# Autodesk Inventor assembly: 00_044_THORAX_YAW_R1
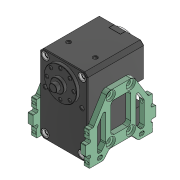
[picture p0: Inventor's stored thumbnail of the model, 180x180]
Saved by Autodesk Inventor 2021.2 (Build 252289000, 289)
## iProperties
Created: 2018-08-06
Part Number: 00_044_THORAX_YAW_R1
Material: 一般
Document SubType Name: Assembly
Designer: student
Mass: 66.6076 g
Surface Area: 177.769 cm^2
Volume: 47.0989 cm^3
Density: 1.41421 g/cm^3
Author: student
## Documents named in this file (4)
- C:\Workspace\HaptHexa\Hardware\Inventor\00_044_THORAX_YAW_R1.iam
- C:\Workspace\HaptHexa\Hardware\Inventor\16_045_THORAX_YAW_FRAME1_R1.ipt
- C:\Workspace\HaptHexa\Hardware\Inventor\20_001_DYNAMIXEL_X430_R1.ipt
- C:\Workspace\HaptHexa\Hardware\Inventor\16_029_X430_FREE_HORN_R1.ipt
## Components (4 placed, 3 different names)
1. yaw_servo_side:1 — Mate:5, Mate:6, Mate:7
2. 20_001_DYNAMIXEL_X430_R1:1 — Flush:1, Flush:2, Mate:1, Insert:1, Mate:5, Mate:6, Mate:7, Mate:8, Mate:9, Mate:10
3. 16_029_X430_FREE_HORN_R1:1 — Insert:1
4. yaw_servo_side:2 — Mate:8, Mate:9, Mate:10
## Relationships (10: Mate 7, Flush 2, Insert 1)
- Flush:1: 20_001_DYNAMIXEL_X430_R1:1
- Flush:2: 20_001_DYNAMIXEL_X430_R1:1
- Mate:1: 20_001_DYNAMIXEL_X430_R1:1
- Insert:1: 20_001_DYNAMIXEL_X430_R1:1 ↔ 16_029_X430_FREE_HORN_R1:1
- Mate:5: yaw_servo_side:1 ↔ 20_001_DYNAMIXEL_X430_R1:1
- Mate:6: yaw_servo_side:1 ↔ 20_001_DYNAMIXEL_X430_R1:1
- Mate:7: yaw_servo_side:1 ↔ 20_001_DYNAMIXEL_X430_R1:1
- Mate:8: 20_001_DYNAMIXEL_X430_R1:1 ↔ yaw_servo_side:2
- Mate:9: 20_001_DYNAMIXEL_X430_R1:1 ↔ yaw_servo_side:2
- Mate:10: 20_001_DYNAMIXEL_X430_R1:1 ↔ yaw_servo_side:2
